# Autodesk Inventor assembly: s-assy-scara_link2
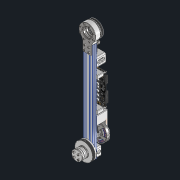
[picture p0: Inventor's stored thumbnail of the model, 180x180]
Saved by Autodesk Inventor 2022 (Build 260153000, 153)
## iProperties
Created: 2021-07-12
Document SubType Name: Assembly
Designer: yuta0
Mass: 1490.4 g
Surface Area: 3935.98 cm^2
Volume: 558.929 cm^3
Density: 2.66653 g/cm^3
Part Number: s-assy-scara_link2
Author: yuta0
## Documents named in this file (15)
- C:\Users\yuta0\Documents\GitHub\catchrobo_hardware\assy-scara\s-assy-scara_link2.iam
- C:\Users\yuta0\Documents\GitHub\catchrobo_hardware\assy-scara\scara-base5.ipt
- C:\Users\yuta0\Documents\GitHub\catchrobo_hardware\assy-scara\KNFS5-2040_2.ipt
- C:\Users\yuta0\Documents\GitHub\catchrobo_hardware\assy-scara\scara-base6.ipt
- C:\Users\yuta0\Documents\GitHub\catchrobo_hardware\assy-scara\scara-belt3.ipt
- C:\Users\yuta0\Documents\GitHub\catchrobo_hardware\assy-scara\s-assy-j3.iam
- C:\Users\yuta0\Documents\GitHub\catchrobo_hardware\assy-scara\HNTT5-5.ipt
- C:\Users\yuta0\Documents\GitHub\catchrobo_hardware\assy-scara\s-assy-outer.iam
- C:\Users\yuta0\Documents\GitHub\catchrobo_hardware\assy-scara\s-assy-odrive.iam
- C:\Users\yuta0\Documents\GitHub\catchrobo_hardware\assy-scara\scara-plate2.ipt
- C:\Users\yuta0\Documents\GitHub\catchrobo_hardware\assy-scara\scara-base14.ipt
- C:\Users\yuta0\Documents\GitHub\catchrobo_hardware\assy-scara\scara-base19.ipt
- C:\Users\yuta0\Documents\GitHub\catchrobo_hardware\assy-scara\scara-base23.ipt
- C:\Users\yuta0\Documents\GitHub\catchrobo_hardware\assy-scara\CB5-55.ipt
- C:\Users\yuta0\Documents\GitHub\catchrobo_hardware\assy-robot\s-assy-unit-j3.iam
## Components (20 placed, 13 different names)
1. scara-base5:1 — メイト:223, メイト:225, メイト:226, メイト:227, メイト:230, メイト:256, メイト:259, メイト:260, メイト:261, メイト:272
2. KNFS5-2040_2:2 — フラッシュ:3, メイト:207, メイト:223, メイト:225, メイト:226, メイト:246, フラッシュ:7, メイト:251, メイト:253, メイト:254, フラッシュ:8, メイト:257, メイト:258, メイト:269, フラッシュ:9, メイト:273
3. scara-base6:1 — メイト:230, メイト:263, メイト:267, メイト:274, メイト:278, メイト:279, メイト:280, メイト:281
4. scara-belt3:1 — メイト:247, メイト:248, メイト:255
5. s-assy-j3:1 [sub-assembly] — メイト:246, メイト:247, フラッシュ:7, メイト:248
6. s-assy-outer:1 [sub-assembly] — メイト:253, メイト:254, フラッシュ:8, メイト:255, メイト:256, メイト:270
7. s-assy-odrive:1 [sub-assembly] — メイト:257, メイト:258
8. scara-plate2:1 — メイト:259, メイト:260, メイト:261, メイト:263, メイト:267
9. scara-plate2:2 — メイト:274, メイト:275, メイト:277, メイト:278, メイト:279
10. scara-base14:1 — メイト:269, フラッシュ:9, メイト:270, フラッシュ:10
11. scara-base19:1 — フラッシュ:10, メイト:272, メイト:273
12. scara-base23:1 — メイト:275, メイト:277, メイト:280, メイト:282
13. CB5-55:1 — メイト:281, メイト:282
14. HNTT5-5:1 — メイト:251
15. CB5-55:2
16. HNTT5-5:2
17. CB5-55:3
18. HNTT5-5:3
19. CB5-55:4
20. HNTT5-5:4
## Component patterns: (4 elements, first: CB5-55:1 + HNTT5-5:1)
## Relationships (38: Mate 33, Flush 5)
- フラッシュ:3 [Flush]: KNFS5-2040_2:2
- メイト:207 [Mate]: KNFS5-2040_2:2
- メイト:223 [Mate]: scara-base5:1 ↔ KNFS5-2040_2:2
- メイト:225 [Mate] (-10 mm): scara-base5:1 ↔ KNFS5-2040_2:2
- メイト:226 [Mate] (-10 mm): scara-base5:1 ↔ KNFS5-2040_2:2
- メイト:227 [Mate]: scara-base5:1
- メイト:230 [Mate]: scara-base5:1 ↔ scara-base6:1
- メイト:246 [Mate]: KNFS5-2040_2:2 ↔ s-assy-j3:1
- メイト:247 [Mate]: scara-belt3:1 ↔ s-assy-j3:1
- フラッシュ:7 [Flush]: KNFS5-2040_2:2 ↔ s-assy-j3:1
- メイト:248 [Mate] (0.5 mm): scara-belt3:1 ↔ s-assy-j3:1
- メイト:251 [Mate]: KNFS5-2040_2:2 ↔ HNTT5-5:1
- メイト:253 [Mate]: KNFS5-2040_2:2 ↔ s-assy-outer:1
- メイト:254 [Mate]: KNFS5-2040_2:2 ↔ s-assy-outer:1
- フラッシュ:8 [Flush]: KNFS5-2040_2:2 ↔ s-assy-outer:1
- メイト:255 [Mate]: scara-belt3:1 ↔ s-assy-outer:1
- メイト:256 [Mate] (450 mm): scara-base5:1 ↔ s-assy-outer:1
- メイト:257 [Mate]: KNFS5-2040_2:2 ↔ s-assy-odrive:1
- メイト:258 [Mate]: KNFS5-2040_2:2 ↔ s-assy-odrive:1
- メイト:259 [Mate]: scara-base5:1 ↔ scara-plate2:1
- メイト:260 [Mate]: scara-base5:1 ↔ scara-plate2:1
- メイト:261 [Mate]: scara-base5:1 ↔ scara-plate2:1
- メイト:263 [Mate]: scara-base6:1 ↔ scara-plate2:1
- メイト:267 [Mate]: scara-base6:1 ↔ scara-plate2:1
- メイト:269 [Mate]: KNFS5-2040_2:2 ↔ scara-base14:1
- フラッシュ:9 [Flush]: KNFS5-2040_2:2 ↔ scara-base14:1
- メイト:270 [Mate] (18 mm): s-assy-outer:1 ↔ scara-base14:1
- フラッシュ:10 [Flush]: scara-base14:1 ↔ scara-base19:1
- メイト:272 [Mate] (15 mm): scara-base5:1 ↔ scara-base19:1
- メイト:273 [Mate]: KNFS5-2040_2:2 ↔ scara-base19:1
- メイト:274 [Mate]: scara-base6:1 ↔ scara-plate2:2
- メイト:275 [Mate]: scara-plate2:2 ↔ scara-base23:1
- メイト:277 [Mate]: scara-plate2:2 ↔ scara-base23:1
- メイト:278 [Mate]: scara-base6:1 ↔ scara-plate2:2
- メイト:279 [Mate]: scara-base6:1 ↔ scara-plate2:2
- メイト:280 [Mate]: scara-base6:1 ↔ scara-base23:1
- メイト:281 [Mate]: scara-base6:1 ↔ CB5-55:1
- メイト:282 [Mate]: scara-base23:1 ↔ CB5-55:1
